# Autodesk Inventor assembly: kanure
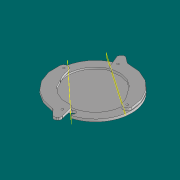
[picture p0: Inventor's stored thumbnail of the model, 180x180]
Saved by Autodesk Inventor 2022 (Build 260153000, 153)
## iProperties
Created: 2023-06-03
Part Number: kanure
Document SubType Name: Assembly
Designer: nyxeon
Author: nyxeon
## Documents named in this file (3)
- C:\Users\gisen\Documents\CAD\inventor\git\cook\canere\canere.iam
- C:\Users\gisen\Documents\CAD\inventor\git\cook\canere\canere_01.ipt
- C:\Users\gisen\Documents\CAD\inventor\git\cook\canere\canere_02_t3_01.ipt
## Components (3 placed, 2 different names)
1. canere_01:1 — メイト:1, メイト:2, メイト:3, メイト:4
2. canere_02_t3_01:1 — メイト:1, メイト:4
3. canere_02_t3_01:2 — メイト:2, メイト:3
## Relationships (4: Mate 4)
- メイト:1 [Mate]: canere_01:1 ↔ canere_02_t3_01:1
- メイト:2 [Mate]: canere_01:1 ↔ canere_02_t3_01:2
- メイト:3 [Mate] (0.5 mm): canere_01:1 ↔ canere_02_t3_01:2
- メイト:4 [Mate] (0.5 mm): canere_01:1 ↔ canere_02_t3_01:1
